# Autodesk Inventor assembly: 4_Camera
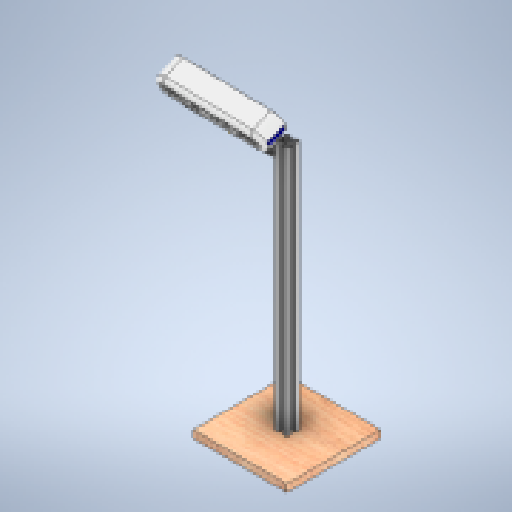
[picture p0: Inventor's stored thumbnail of the model, 512x512]
Saved by Autodesk Inventor 2024 (Build 280153000, 153)
## iProperties
Created: 2023-11-26
Part Number: 4_Camera
Document SubType Name: Assembly
Designer: 박동준
Author: 박동준
## Documents named in this file (5)
- C:\Users\박동준\OneDrive - 연세대학교 (Yonsei University)\바탕 화면\박동준\대학생할\로봇\Humanoid\7축 매니퓰레이터\하드웨어\rh_plus_7_axis_robot_arm_hardware\Assembly\4_Camera.iam
- C:\Users\박동준\OneDrive - 연세대학교 (Yonsei University)\바탕 화면\박동준\대학생할\로봇\Humanoid\7축 매니퓰레이터\하드웨어\rh_plus_7_axis_robot_arm_hardware\Part\Other Parts\Aluminum_Profile_2020_40mm.ipt
- C:\Users\박동준\OneDrive - 연세대학교 (Yonsei University)\바탕 화면\박동준\대학생할\로봇\Humanoid\7축 매니퓰레이터\하드웨어\rh_plus_7_axis_robot_arm_hardware\Part\Other Parts\Aluminum_Profile_2020_15mm.ipt
- C:\Users\박동준\OneDrive - 연세대학교 (Yonsei University)\바탕 화면\박동준\대학생할\로봇\Humanoid\7축 매니퓰레이터\하드웨어\rh_plus_7_axis_robot_arm_hardware\Part\Other Parts\Camera_base_plate.ipt
- C:\Users\박동준\OneDrive - 연세대학교 (Yonsei University)\바탕 화면\박동준\대학생할\로봇\Humanoid\7축 매니퓰레이터\하드웨어\rh_plus_7_axis_robot_arm_hardware\Part\Other Parts\Astra + Camera.ipt
## Components (4 placed, 4 different names)
1. Aluminum_Profile_2020_40mm:1 — Mate:1, Mate:2, Angle:2, Mate:3, Angle:3, Mate:4, Mate:5, Mate:8, Angle:4, Mate:9
2. Aluminum_Profile_2020_15mm:1 — Mate:3, Angle:3, Mate:4, Mate:5, Mate:10, Flush:1, Mate:11
3. Camera_base_plate:1 — Mate:8, Angle:4, Mate:9
4. Astra + Camera:1 — Mate:10, Flush:1, Mate:11
## Relationships (13: Mate 9, Angle 3, Flush 1)
- Mate:1: Aluminum_Profile_2020_40mm:1
- Mate:2: Aluminum_Profile_2020_40mm:1
- Angle:2 (0 deg): Aluminum_Profile_2020_40mm:1
- Mate:3: Aluminum_Profile_2020_40mm:1 ↔ Aluminum_Profile_2020_15mm:1
- Angle:3 (25 deg): Aluminum_Profile_2020_40mm:1 ↔ Aluminum_Profile_2020_15mm:1
- Mate:4: Aluminum_Profile_2020_40mm:1 ↔ Aluminum_Profile_2020_15mm:1
- Mate:5: Aluminum_Profile_2020_40mm:1 ↔ Aluminum_Profile_2020_15mm:1
- Mate:8: Aluminum_Profile_2020_40mm:1 ↔ Camera_base_plate:1
- Angle:4 (0 deg): Aluminum_Profile_2020_40mm:1 ↔ Camera_base_plate:1
- Mate:9: Aluminum_Profile_2020_40mm:1 ↔ Camera_base_plate:1
- Mate:10: Aluminum_Profile_2020_15mm:1 ↔ Astra + Camera:1
- Flush:1 (13 mm): Aluminum_Profile_2020_15mm:1 ↔ Astra + Camera:1
- Mate:11: Aluminum_Profile_2020_15mm:1 ↔ Astra + Camera:1
